# Autodesk Inventor assembly: ModulKolaNapinajacego
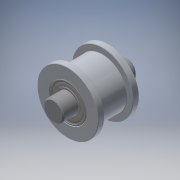
[picture p0: Inventor's stored thumbnail of the model, 180x180]
Saved by Autodesk Inventor 2019 (Build 230136000, 136)
## iProperties
Created: 2020-05-23
Part Number: ModulKolaNapinajacego
Document SubType Name: Assembly
Designer: estee
Author: estee
## Documents named in this file (3)
- C:\Users\estee\OneDrive\Pulpit\estere\1\MUM\projejt\ModulKolaNapinajacego.iam
- C:\Users\estee\OneDrive\Pulpit\estere\1\MUM\projejt\walekpodkolonapinajace.ipt
- C:\Users\estee\OneDrive\Pulpit\estere\1\MUM\projejt\Gates_2GT_20T_Smooth_Idler.ipt
## Components (2 placed, 2 different names)
1. walekpodkolonapinajace:1 — Mate:1
2. Gates_2GT_20T_Smooth_Idler:1 — Mate:1
## Relationships (1: Mate 1)
- Mate:1: walekpodkolonapinajace:1 ↔ Gates_2GT_20T_Smooth_Idler:1
